# Autodesk Inventor assembly: FullWheelAJB
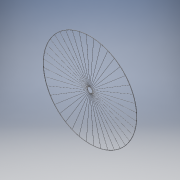
[picture p0: Inventor's stored thumbnail of the model, 180x180]
Saved by Autodesk Inventor 2018 (Build 220112000, 112)
## iProperties
Created: 2018-01-18
Part Number: FullWheelAJB
Document SubType Name: Assembly
Designer: Alec temporary
Author: Alec temporary
## Documents named in this file (3)
- C:\Users\Alec temporary\Desktop\New folder\FullWheelAJB.iam
- C:\Users\Alec temporary\Desktop\New folder\1_40th_WheelAJB.ipt
- C:\Users\Alec temporary\Desktop\New folder\InnerWheelAJB.ipt
## Components (41 placed, 2 different names)
1. InnerWheelAJB:1 — Flush:1, Flush:2
2. 1_40th_WheelAJB:1
3. 1_40th_WheelAJB:2
4. 1_40th_WheelAJB:3
5. 1_40th_WheelAJB:4
6. 1_40th_WheelAJB:5
7. 1_40th_WheelAJB:6
8. 1_40th_WheelAJB:7
9. 1_40th_WheelAJB:8
10. 1_40th_WheelAJB:9
11. 1_40th_WheelAJB:10
12. 1_40th_WheelAJB:11
13. 1_40th_WheelAJB:12
14. 1_40th_WheelAJB:13
15. 1_40th_WheelAJB:14
16. 1_40th_WheelAJB:15
17. 1_40th_WheelAJB:16
18. 1_40th_WheelAJB:17
19. 1_40th_WheelAJB:18
20. 1_40th_WheelAJB:19 — Flush:1
21. 1_40th_WheelAJB:20
22. 1_40th_WheelAJB:21 — Flush:2
23. 1_40th_WheelAJB:22
24. 1_40th_WheelAJB:23
25. 1_40th_WheelAJB:24
26. 1_40th_WheelAJB:25
27. 1_40th_WheelAJB:26
28. 1_40th_WheelAJB:27
29. 1_40th_WheelAJB:28
30. 1_40th_WheelAJB:29
31. 1_40th_WheelAJB:30
32. 1_40th_WheelAJB:31
33. 1_40th_WheelAJB:32
34. 1_40th_WheelAJB:33
35. 1_40th_WheelAJB:34
36. 1_40th_WheelAJB:35
37. 1_40th_WheelAJB:36
38. 1_40th_WheelAJB:37
39. 1_40th_WheelAJB:38
40. 1_40th_WheelAJB:39
41. 1_40th_WheelAJB:40
## Component patterns: (40 elements, first: 1_40th_WheelAJB:1)
## Relationships (2: Flush 2)
- Flush:1: InnerWheelAJB:1 ↔ 1_40th_WheelAJB:19
- Flush:2: InnerWheelAJB:1 ↔ 1_40th_WheelAJB:21
